# Autodesk Inventor assembly: Phone assembly solution
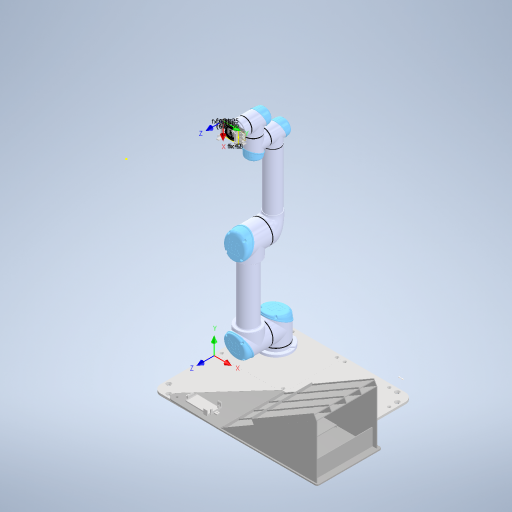
[picture p0: Inventor's stored thumbnail of the model, 512x512]
Saved by Autodesk Inventor 2024 (Build 280153000, 153)
## iProperties
Created: 2024-03-26
Part Number: Phone assembly solution
Document SubType Name: Assembly
Designer: jens1
Author: jens1
## Documents named in this file (14)
- C:\Users\jens1\Documents\GitHub\Robotteknologi-2.-semester\3D modeller\Phone assembly solution.iam
- C:\Users\jens1\Documents\GitHub\Robotteknologi-2.-semester\3D modeller\UR5\UR5\UR5.iam
- C:\Users\jens1\Documents\GitHub\Robotteknologi-2.-semester\3D modeller\Mount plate UR.ipt
- C:\Users\jens1\Documents\GitHub\Robotteknologi-2.-semester\3D modeller\Left bottom plate.ipt
- C:\Users\jens1\Documents\GitHub\Robotteknologi-2.-semester\3D modeller\Right bottom plate.ipt
- C:\Users\jens1\Documents\GitHub\Robotteknologi-2.-semester\3D modeller\Right top plate.ipt
- C:\Users\jens1\Documents\GitHub\Robotteknologi-2.-semester\3D modeller\Phone\Sikring.ipt
- C:\Users\jens1\Documents\GitHub\Robotteknologi-2.-semester\3D modeller\Gripper\Gripper.iam
- C:\Users\jens1\Documents\GitHub\Robotteknologi-2.-semester\3D modeller\Phone\Bund.ipt
- C:\Users\jens1\Documents\GitHub\Robotteknologi-2.-semester\3D modeller\Phone\Top.ipt
- C:\Users\jens1\Documents\GitHub\Robotteknologi-2.-semester\3D modeller\Phone\PCB.ipt
- C:\Users\jens1\Documents\GitHub\Robotteknologi-2.-semester\3D modeller\Mounting station.ipt
- C:\Users\jens1\Documents\GitHub\Robotteknologi-2.-semester\3D modeller\Input\Configuration 2.ipt
- C:\Users\jens1\Documents\GitHub\Robotteknologi-2.-semester\3D modeller\Input\Boltplade v2.ipt
## Components (13 placed, 13 different names)
1. UR5:1 [sub-assembly] — Mate:2, Mate:3, Mate:4, Tangent:1, Mate:9, Mate:10, Mate:11
2. Mount plate UR:1 — Mate:1, Mate:2, Mate:3, Mate:4, Tangent:1, Flush:1, Mate:5, Flush:2, Flush:5, Mate:8
3. Left bottom plate:1 — Flush:1, Mate:5, Flush:2, Flush:3, Mate:6, Flush:4, Mate:14
4. Right bottom plate:1 — Flush:3, Mate:6, Flush:4, Mate:7, Mate:13, Flush:7
5. Right top plate:1 — Flush:5, Mate:7, Mate:8
6. Gripper:1 [sub-assembly] — Mate:9, Mate:10, Mate:11
7. Sikring:2
8. Bund:1
9. Top:1 — Mate:12, Tangent:2, Flush:6
10. PCB:1 — Mate:12, Tangent:2, Flush:6
11. Mounting station:1 — Mate:18, Mate:19, Mate:20
12. Boltplade v2:1 — Mate:13, Mate:14, Flush:7, Mate:15, Mate:16, Mate:17, Mate:18, Mate:19, Mate:20
13. Configuration 2:1 — Mate:15, Mate:16, Mate:17
## Relationships (29: Mate 20, Flush 7, Tangent 2)
- Mate:1: Mount plate UR:1
- Mate:2: UR5:1 ↔ Mount plate UR:1
- Mate:3 (-116 mm): UR5:1 ↔ Mount plate UR:1
- Mate:4 (-116 mm): UR5:1 ↔ Mount plate UR:1
- Tangent:1 (0.25 mm): UR5:1 ↔ Mount plate UR:1
- Flush:1: Mount plate UR:1 ↔ Left bottom plate:1
- Mate:5: Mount plate UR:1 ↔ Left bottom plate:1
- Flush:2: Mount plate UR:1 ↔ Left bottom plate:1
- Flush:3: Left bottom plate:1 ↔ Right bottom plate:1
- Mate:6: Left bottom plate:1 ↔ Right bottom plate:1
- Flush:4: Left bottom plate:1 ↔ Right bottom plate:1
- Flush:5: Mount plate UR:1 ↔ Right top plate:1
- Mate:7: Right bottom plate:1 ↔ Right top plate:1
- Mate:8: Mount plate UR:1 ↔ Right top plate:1
- Mate:9: UR5:1 ↔ Gripper:1
- Mate:10: UR5:1 ↔ Gripper:1
- Mate:11: UR5:1 ↔ Gripper:1
- Mate:12: Top:1 ↔ PCB:1
- Tangent:2 (3.5 mm): Top:1 ↔ PCB:1
- Flush:6 (18.25 mm): Top:1 ↔ PCB:1
- Mate:13: Right bottom plate:1 ↔ Boltplade v2:1
- Mate:14: Left bottom plate:1 ↔ Boltplade v2:1
- Flush:7 (142.216 mm): Right bottom plate:1 ↔ Boltplade v2:1
- Mate:15: Boltplade v2:1 ↔ Configuration 2:1
- Mate:16: Boltplade v2:1 ↔ Configuration 2:1
- Mate:17: Boltplade v2:1 ↔ Configuration 2:1
- Mate:18: Mounting station:1 ↔ Boltplade v2:1
- Mate:19: Mounting station:1 ↔ Boltplade v2:1
- Mate:20 (5.5 mm): Mounting station:1 ↔ Boltplade v2:1
